# Autodesk Inventor assembly: YY
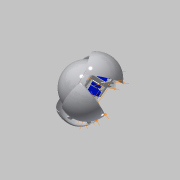
[picture p0: Inventor's stored thumbnail of the model, 180x180]
Saved by Autodesk Inventor 2020 (Build 240168000, 168)
## iProperties
Created: 2019-02-07
Part Number: YY
Material: Generisch
Document SubType Name: Assembly
Designer: Lion
Mass: 376.84 g
Surface Area: 1844.42 cm^2
Volume: 210.973 cm^3
Density: 1.7862 g/cm^3
Author: Lion
## Documents named in this file (17)
- D:\Projects\Rollbot\YY.iam
- D:\Projects\Rollbot\BaseBottom.ipt
- D:\Projects\Rollbot\BaseTop.ipt
- D:\Projects\Rollbot\Servo Motor SG90.ipt
- D:\Projects\Rollbot\PlaceholderSmall.ipt
- D:\Projects\Rollbot\PlaceholderLarge.ipt
- D:\Users\Lion\Documents\Inventor\Content Center Files\R2019\de-DE\DIN 84\DIN 84 - M2 x 20.ipt
- D:\Users\Lion\Documents\Inventor\Content Center Files\R2019\de-DE\DIN 84\DIN 84 - M2 x 12.ipt
- D:\Users\Lion\Documents\Inventor\Content Center Files\R2019\de-DE\DIN 934\DIN 934 - M2 x 0.4.ipt
- D:\Projects\Rollbot\LegBase.ipt
- D:\Projects\Rollbot\LegRightLarge.ipt
- D:\Projects\Rollbot\ShellLower.ipt
- D:\Projects\Rollbot\ShaftLegLower.ipt
- D:\Projects\Rollbot\LegConnector.ipt
- D:\Projects\Rollbot\ShaftLegUpper.ipt
- D:\Projects\Rollbot\TopConnector.ipt
- D:\Projects\Rollbot\ShellTop.ipt
## Components (68 placed, 16 different names)
1. BaseBottom:1 — Einfügen:1, Einfügen:2, Einfügen:3, Einfügen:4, Einfügen:5, Einfügen:6, Einfügen:7, Einfügen:8, Einfügen:21, Einfügen:22, Einfügen:23, Einfügen:24, Einfügen:25, Einfügen:26, Einfügen:27, Einfügen:28, Passend:13
2. BaseTop:1 — Einfügen:29, Einfügen:30, Einfügen:31, Einfügen:32, Einfügen:33, Einfügen:34, Einfügen:35, Einfügen:36, WinkelBase, Winkel:3, Winkel:5, Winkel:7, Passend:11, Passend:12
3. Servo Motor SG90:1 — Einfügen:12, Einfügen:16, Einfügen:20, Passend:10, Einfügen:67
4. Servo Motor SG90:2 — Einfügen:10, Einfügen:14, Einfügen:17, Passend:6, Einfügen:47
5. Servo Motor SG90:3 — Einfügen:11, Einfügen:15, Einfügen:18, Passend:4, Einfügen:37
6. Servo Motor SG90:4 — Einfügen:9, Einfügen:13, Einfügen:19, Passend:8, Einfügen:57
7. PlaceholderSmall:1 — Einfügen:2, Einfügen:11
8. PlaceholderSmall:2 — Einfügen:6, Einfügen:10
9. PlaceholderSmall:3 — Einfügen:7, Einfügen:15
10. PlaceholderSmall:4 — Einfügen:5, Einfügen:9
11. PlaceholderSmall:5 — Einfügen:3, Einfügen:12
12. PlaceholderSmall:6 — Einfügen:4, Einfügen:13
13. PlaceholderSmall:7 — Einfügen:1, Einfügen:16
14. PlaceholderSmall:8 — Einfügen:8, Einfügen:14
15. PlaceholderLarge:1 — Einfügen:17, Einfügen:30
16. PlaceholderLarge:2 — Einfügen:18, Einfügen:31
17. PlaceholderLarge:3 — Einfügen:20, Einfügen:32
18. PlaceholderLarge:4 — Einfügen:19, Einfügen:29
19. DIN 84 - ersetzt durch DIN EN ISO 1207 M2 x 20:1 — Einfügen:21
20. DIN 84 - ersetzt durch DIN EN ISO 1207 M2 x 20:2 — Einfügen:22
21. DIN 84 - ersetzt durch DIN EN ISO 1207 M2 x 20:3 — Einfügen:23
22. DIN 84 - ersetzt durch DIN EN ISO 1207 M2 x 20:4 — Einfügen:24
23. DIN 84 - ersetzt durch DIN EN ISO 1207 M2 x 12:1 — Einfügen:25, Passend:3
24. DIN 84 - ersetzt durch DIN EN ISO 1207 M2 x 12:2 — Einfügen:28, Passend:5
25. DIN 84 - ersetzt durch DIN EN ISO 1207 M2 x 12:3 — Einfügen:27, Passend:7
26. DIN 84 - ersetzt durch DIN EN ISO 1207 M2 x 12:4 — Einfügen:26, Passend:9
27. DIN 934 - ersetzt durch DIN EN 24032/28673/28674 M2:1 — Passend:3, Passend:4
28. DIN 934 - ersetzt durch DIN EN 24032/28673/28674 M2:2 — Passend:5, Passend:6
29. DIN 934 - ersetzt durch DIN EN 24032/28673/28674 M2:3 — Passend:7, Passend:8
30. DIN 934 - ersetzt durch DIN EN 24032/28673/28674 M2:4 — Passend:9, Passend:10
31. DIN 934 - ersetzt durch DIN EN 24032/28673/28674 M2:5 — Einfügen:33
32. DIN 934 - ersetzt durch DIN EN 24032/28673/28674 M2:6 — Einfügen:34
33. DIN 934 - ersetzt durch DIN EN 24032/28673/28674 M2:7 — Einfügen:35
34. DIN 934 - ersetzt durch DIN EN 24032/28673/28674 M2:8 — Einfügen:36
35. LegBase:1 — Einfügen:37, Einfügen:38, Einfügen:39, WinkelBase, WinkelConnector, Einfügen:43, Einfügen:45
36. Servo Motor SG90:5 — Einfügen:38, Einfügen:39, Einfügen:40
37. LegBottom:1 — Einfügen:40, WinkelConnector, Einfügen:42
38. ShellLower:1 — Einfügen:41, Einfügen:42, Einfügen:44
39. ShaftLegLower:1 — Einfügen:41
40. LegConnector:1 — Einfügen:43, Einfügen:44, Einfügen:46
41. ShaftLegUpper:1 — Einfügen:45
42. ShaftLegUpper:2 — Einfügen:46
43. LegBase:2 — Einfügen:47, Winkel:3, Einfügen:48, Einfügen:49, Winkel:4, Einfügen:53, Einfügen:55
44. Servo Motor SG90:6 — Einfügen:48, Einfügen:49, Einfügen:50
45. LegBottom:2 — Einfügen:50, Winkel:4, Einfügen:51
46. ShellLower:2 — Einfügen:51, Einfügen:52, Einfügen:54
47. ShaftLegLower:2 — Einfügen:52
48. LegConnector:2 — Einfügen:53, Einfügen:54, Einfügen:56
49. ShaftLegUpper:3 — Einfügen:55
50. ShaftLegUpper:4 — Einfügen:56
51. LegBase:3 — Einfügen:57, Winkel:5, Einfügen:58, Einfügen:59, Winkel:6, Einfügen:63
52. Servo Motor SG90:7 — Einfügen:58, Einfügen:59, Einfügen:60
53. LegBottom:3 — Einfügen:60, Winkel:6, Einfügen:61
54. ShellLower:3 — Einfügen:61, Einfügen:62, Einfügen:64
55. ShaftLegLower:3 — Einfügen:62
56. LegConnector:3 — Einfügen:63, Einfügen:64, Einfügen:65, Einfügen:66
57. ShaftLegUpper:5 — Einfügen:65
58. ShaftLegUpper:6 — Einfügen:66
59. LegBase:4 — Einfügen:67, Winkel:7, Einfügen:68, Einfügen:69, Winkel:8, Einfügen:73, Einfügen:76
60. Servo Motor SG90:8 — Einfügen:68, Einfügen:69, Einfügen:70
61. ShellLower:4 — Einfügen:71, Einfügen:72, Einfügen:74
62. LegBottom:4 — Einfügen:70, Winkel:8, Einfügen:71
63. ShaftLegLower:4 — Einfügen:72
64. LegConnector:4 — Einfügen:73, Einfügen:74, Einfügen:75
65. ShaftLegUpper:7 — Einfügen:75
66. ShaftLegUpper:8 — Einfügen:76
67. TopConnector:1 — Passend:11, Passend:12, Passend:13, Passend:14, Fluchtend:1, Fluchtend:2
68. ShellTop:1 — Passend:14, Fluchtend:1, Fluchtend:2
## Relationships (98: Insert 76, Mate 12, Angle 8, Flush 2)
- Einfügen:1 [Insert]: BaseBottom:1 ↔ PlaceholderSmall:7
- Einfügen:2 [Insert]: BaseBottom:1 ↔ PlaceholderSmall:1
- Einfügen:3 [Insert]: BaseBottom:1 ↔ PlaceholderSmall:5
- Einfügen:4 [Insert]: BaseBottom:1 ↔ PlaceholderSmall:6
- Einfügen:5 [Insert]: BaseBottom:1 ↔ PlaceholderSmall:4
- Einfügen:6 [Insert]: BaseBottom:1 ↔ PlaceholderSmall:2
- Einfügen:7 [Insert]: BaseBottom:1 ↔ PlaceholderSmall:3
- Einfügen:8 [Insert]: BaseBottom:1 ↔ PlaceholderSmall:8
- Einfügen:9 [Insert]: Servo Motor SG90:4 ↔ PlaceholderSmall:4
- Einfügen:10 [Insert]: Servo Motor SG90:2 ↔ PlaceholderSmall:2
- Einfügen:11 [Insert]: Servo Motor SG90:3 ↔ PlaceholderSmall:1
- Einfügen:12 [Insert]: Servo Motor SG90:1 ↔ PlaceholderSmall:5
- Einfügen:13 [Insert]: Servo Motor SG90:4 ↔ PlaceholderSmall:6
- Einfügen:14 [Insert]: Servo Motor SG90:2 ↔ PlaceholderSmall:8
- Einfügen:15 [Insert]: Servo Motor SG90:3 ↔ PlaceholderSmall:3
- Einfügen:16 [Insert]: Servo Motor SG90:1 ↔ PlaceholderSmall:7
- Einfügen:17 [Insert]: Servo Motor SG90:2 ↔ PlaceholderLarge:1
- Einfügen:18 [Insert]: Servo Motor SG90:3 ↔ PlaceholderLarge:2
- Einfügen:19 [Insert]: Servo Motor SG90:4 ↔ PlaceholderLarge:4
- Einfügen:20 [Insert]: Servo Motor SG90:1 ↔ PlaceholderLarge:3
- Einfügen:21 [Insert]: BaseBottom:1 ↔ DIN 84 - ersetzt durch DIN EN ISO 1207 M2 x 20:1
- Einfügen:22 [Insert]: BaseBottom:1 ↔ DIN 84 - ersetzt durch DIN EN ISO 1207 M2 x 20:2
- Einfügen:23 [Insert]: BaseBottom:1 ↔ DIN 84 - ersetzt durch DIN EN ISO 1207 M2 x 20:3
- Einfügen:24 [Insert]: BaseBottom:1 ↔ DIN 84 - ersetzt durch DIN EN ISO 1207 M2 x 20:4
- Einfügen:25 [Insert]: BaseBottom:1 ↔ DIN 84 - ersetzt durch DIN EN ISO 1207 M2 x 12:1
- Einfügen:26 [Insert]: BaseBottom:1 ↔ DIN 84 - ersetzt durch DIN EN ISO 1207 M2 x 12:4
- Einfügen:27 [Insert]: BaseBottom:1 ↔ DIN 84 - ersetzt durch DIN EN ISO 1207 M2 x 12:3
- Einfügen:28 [Insert]: BaseBottom:1 ↔ DIN 84 - ersetzt durch DIN EN ISO 1207 M2 x 12:2
- Einfügen:29 [Insert]: BaseTop:1 ↔ PlaceholderLarge:4
- Einfügen:30 [Insert]: BaseTop:1 ↔ PlaceholderLarge:1
- Einfügen:31 [Insert]: BaseTop:1 ↔ PlaceholderLarge:2
- Einfügen:32 [Insert]: BaseTop:1 ↔ PlaceholderLarge:3
- Passend:3 [Mate]: DIN 84 - ersetzt durch DIN EN ISO 1207 M2 x 12:1 ↔ DIN 934 - ersetzt durch DIN EN 24032/28673/28674 M2:1
- Passend:4 [Mate]: Servo Motor SG90:3 ↔ DIN 934 - ersetzt durch DIN EN 24032/28673/28674 M2:1
- Passend:5 [Mate]: DIN 84 - ersetzt durch DIN EN ISO 1207 M2 x 12:2 ↔ DIN 934 - ersetzt durch DIN EN 24032/28673/28674 M2:2
- Passend:6 [Mate]: Servo Motor SG90:2 ↔ DIN 934 - ersetzt durch DIN EN 24032/28673/28674 M2:2
- Passend:7 [Mate]: DIN 84 - ersetzt durch DIN EN ISO 1207 M2 x 12:3 ↔ DIN 934 - ersetzt durch DIN EN 24032/28673/28674 M2:3
- Passend:8 [Mate]: Servo Motor SG90:4 ↔ DIN 934 - ersetzt durch DIN EN 24032/28673/28674 M2:3
- Passend:9 [Mate]: DIN 84 - ersetzt durch DIN EN ISO 1207 M2 x 12:4 ↔ DIN 934 - ersetzt durch DIN EN 24032/28673/28674 M2:4
- Passend:10 [Mate]: Servo Motor SG90:1 ↔ DIN 934 - ersetzt durch DIN EN 24032/28673/28674 M2:4
- Einfügen:33 [Insert]: BaseTop:1 ↔ DIN 934 - ersetzt durch DIN EN 24032/28673/28674 M2:5
- Einfügen:34 [Insert]: BaseTop:1 ↔ DIN 934 - ersetzt durch DIN EN 24032/28673/28674 M2:6
- Einfügen:35 [Insert]: BaseTop:1 ↔ DIN 934 - ersetzt durch DIN EN 24032/28673/28674 M2:7
- Einfügen:36 [Insert]: BaseTop:1 ↔ DIN 934 - ersetzt durch DIN EN 24032/28673/28674 M2:8
- Einfügen:37 [Insert] (-1.5 mm): Servo Motor SG90:3 ↔ LegBase:1
- Einfügen:38 [Insert]: LegBase:1 ↔ Servo Motor SG90:5
- Einfügen:39 [Insert]: LegBase:1 ↔ Servo Motor SG90:5
- Einfügen:40 [Insert] (-1.5 mm): Servo Motor SG90:5 ↔ LegBottom:1
- WinkelBase [Angle] (50 deg): BaseTop:1 ↔ LegBase:1
- WinkelConnector [Angle] (-40 deg): LegBase:1 ↔ LegBottom:1
- Einfügen:41 [Insert] (-2.5 mm): ShellLower:1 ↔ ShaftLegLower:1
- Einfügen:42 [Insert] (0.25 mm): LegBottom:1 ↔ ShellLower:1
- Einfügen:43 [Insert] (0.5 mm): LegBase:1 ↔ LegConnector:1
- Einfügen:44 [Insert] (0.5 mm): ShellLower:1 ↔ LegConnector:1
- Einfügen:45 [Insert] (-3 mm): LegBase:1 ↔ ShaftLegUpper:1
- Einfügen:46 [Insert] (-3.5 mm): LegConnector:1 ↔ ShaftLegUpper:2
- Einfügen:47 [Insert] (-2 mm): Servo Motor SG90:2 ↔ LegBase:2
- Winkel:3 [Angle] (50 deg): BaseTop:1 ↔ LegBase:2
- Einfügen:48 [Insert]: LegBase:2 ↔ Servo Motor SG90:6
- Einfügen:49 [Insert]: LegBase:2 ↔ Servo Motor SG90:6
- Einfügen:50 [Insert] (-2 mm): Servo Motor SG90:6 ↔ LegBottom:2
- Winkel:4 [Angle] (-40 deg): LegBase:2 ↔ LegBottom:2
- Einfügen:51 [Insert] (0.25 mm): LegBottom:2 ↔ ShellLower:2
- Einfügen:52 [Insert] (-2.5 mm): ShellLower:2 ↔ ShaftLegLower:2
- Einfügen:53 [Insert] (0.5 mm): LegBase:2 ↔ LegConnector:2
- Einfügen:54 [Insert] (0.5 mm): ShellLower:2 ↔ LegConnector:2
- Einfügen:55 [Insert] (-3 mm): LegBase:2 ↔ ShaftLegUpper:3
- Einfügen:56 [Insert] (-3.5 mm): LegConnector:2 ↔ ShaftLegUpper:4
- Einfügen:57 [Insert] (-2 mm): Servo Motor SG90:4 ↔ LegBase:3
- Winkel:5 [Angle] (50 deg): BaseTop:1 ↔ LegBase:3
- Einfügen:58 [Insert]: LegBase:3 ↔ Servo Motor SG90:7
- Einfügen:59 [Insert]: LegBase:3 ↔ Servo Motor SG90:7
- Einfügen:60 [Insert] (-2 mm): Servo Motor SG90:7 ↔ LegBottom:3
- Winkel:6 [Angle] (-40 deg): LegBase:3 ↔ LegBottom:3
- Einfügen:61 [Insert] (0.25 mm): LegBottom:3 ↔ ShellLower:3
- Einfügen:62 [Insert] (-2.5 mm): ShellLower:3 ↔ ShaftLegLower:3
- Einfügen:63 [Insert] (0.5 mm): LegBase:3 ↔ LegConnector:3
- Einfügen:64 [Insert] (0.5 mm): ShellLower:3 ↔ LegConnector:3
- Einfügen:65 [Insert] (-3 mm): LegConnector:3 ↔ ShaftLegUpper:5
- Einfügen:66 [Insert] (-3.5 mm): LegConnector:3 ↔ ShaftLegUpper:6
- Einfügen:67 [Insert] (-2 mm): Servo Motor SG90:1 ↔ LegBase:4
- Winkel:7 [Angle] (50 deg): BaseTop:1 ↔ LegBase:4
- Einfügen:68 [Insert]: LegBase:4 ↔ Servo Motor SG90:8
- Einfügen:69 [Insert]: LegBase:4 ↔ Servo Motor SG90:8
- Einfügen:70 [Insert] (-2 mm): Servo Motor SG90:8 ↔ LegBottom:4
- Winkel:8 [Angle] (-40 deg): LegBase:4 ↔ LegBottom:4
- Einfügen:71 [Insert] (0.25 mm): ShellLower:4 ↔ LegBottom:4
- Einfügen:72 [Insert] (-2.5 mm): ShellLower:4 ↔ ShaftLegLower:4
- Einfügen:73 [Insert] (0.5 mm): LegBase:4 ↔ LegConnector:4
- Einfügen:74 [Insert] (0.5 mm): ShellLower:4 ↔ LegConnector:4
- Einfügen:75 [Insert] (-3.5 mm): LegConnector:4 ↔ ShaftLegUpper:7
- Einfügen:76 [Insert] (-3 mm): LegBase:4 ↔ ShaftLegUpper:8
- Passend:11 [Mate]: BaseTop:1 ↔ TopConnector:1
- Passend:12 [Mate]: BaseTop:1 ↔ TopConnector:1
- Passend:13 [Mate] (2.5 mm): BaseBottom:1 ↔ TopConnector:1
- Passend:14 [Mate] (0.5 mm): TopConnector:1 ↔ ShellTop:1
- Fluchtend:1 [Flush]: TopConnector:1 ↔ ShellTop:1
- Fluchtend:2 [Flush]: TopConnector:1 ↔ ShellTop:1
## Named parameters: angle_base = 50 deg, angle_connector = -40 deg
